# Autodesk Inventor assembly: combined_mounts_v1
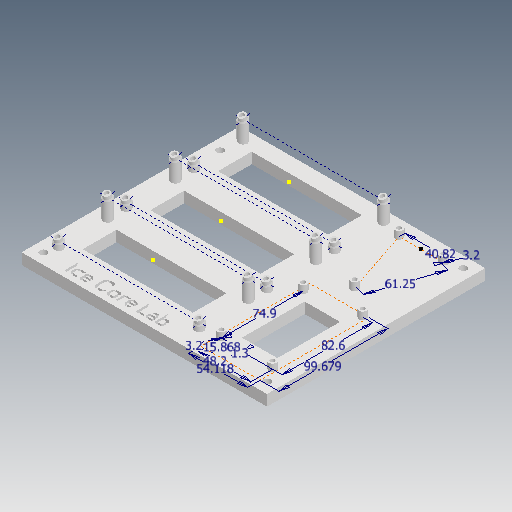
[picture p0: Inventor's stored thumbnail of the model, 512x512]
Saved by Autodesk Inventor 2025.1 (Build 291241000, 241)
## iProperties
Created: 2026-06-20
Part Number: combined_mounts_v1
Document SubType Name: Assembly
Designer: Aiden
Author: Aiden
## Documents named in this file (5)
- C:\Users\Aiden\Documents\GitHub\coldex-instrumentation\hardware\mounting_hardware\mounting_plate_mega_v1.iam
- C:\Users\Aiden\Documents\GitHub\coldex-instrumentation\hardware\mounting_hardware\base_plate.ipt
- C:\Users\Aiden\Documents\GitHub\coldex-instrumentation\hardware\mounting_hardware\arduino_mega_standoffs.ipt
- C:\Users\Aiden\Documents\GitHub\coldex-instrumentation\hardware\mounting_hardware\relay_module_standoffs_angled.ipt
- C:\Users\Aiden\Documents\GitHub\coldex-instrumentation\hardware\mounting_hardware\db-25_standoffs.ipt
## Components (6 placed, 4 different names)
1. base_plate:1 — Mate:2, Mate:5, Mate:6
2. arduino_mega_standoffs:1 — Mate:5
3. db-25_standoffs:1 — Mate:6
4. relay_module_standoffs_angled:1 — Mate:2
5. relay_module_standoffs_angled:2
6. relay_module_standoffs_angled:3
## Component patterns: (3 elements, first: relay_module_standoffs_angled:1)
## Relationships (3: Mate 3)
- Mate:2: base_plate:1 ↔ relay_module_standoffs_angled:1
- Mate:5: base_plate:1 ↔ arduino_mega_standoffs:1
- Mate:6: base_plate:1 ↔ db-25_standoffs:1
